# Autodesk Inventor assembly: X Axis Assembly
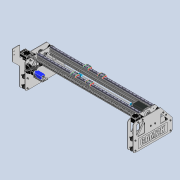
[picture p0: Inventor's stored thumbnail of the model, 180x180]
Saved by Autodesk Inventor 2022 (Build 260153000, 153)
## iProperties
Created: 2021-10-14
Part Number: X Axis Assembly
Document SubType Name: Assembly
Designer: Coy
Author: Coy
## Documents named in this file (35)
- H:\3D Files\Project 3D Models\Breakfast Maker 2000\Assemblys\X Axis Assembly.iam
- H:\3D Files\Project 3D Models\Breakfast Maker 2000\Aluminum Extrusion\2040\2040x700 silver profile.ipt
- H:\3D Files\Project 3D Models\Breakfast Maker 2000\Motors\Nema 23 Dual Shaft 87mm Stepper Motor.ipt
- H:\3D Files\Project 3D Models\Breakfast Maker 2000\Couplers\M6.35 Rigid Coupler.ipt
- H:\3D Files\Project 3D Models\Breakfast Maker 2000\Shafts and Rods\M6.35 x 356mm Aluminum Rod.ipt
- H:\3D Files\Project 3D Models\Breakfast Maker 2000\Linear Actuators\MGN12C Linear Rail.iam
- H:\3D Files\Downloaded 3D Files\GrabCad Downloads\hiwin-mgn-series-full-2.snapshot.14\PRODUCT_NAME_10.ipt
- H:\3D Files\Project 3D Models\Breakfast Maker 2000\Pullys\M6.35 24Tooth 15mm Deep 3M Timing Pulley.ipt
- H:\3D Files\Project 3D Models\Breakfast Maker 2000\Shafts and Rods\M5 55mm Threaded Rod.ipt
- H:\3D Files\Project 3D Models\Breakfast Maker 2000\Nuts and Bolts\M5 Nut Silver.ipt
- H:\3D Files\Project 3D Models\Breakfast Maker 2000\3D Printed Parts\Idler Pully Spacer.ipt
- H:\3D Files\Project 3D Models\Breakfast Maker 2000\3D Printed Parts\V Wheel Spacer.ipt
- H:\3D Files\Project 3D Models\Breakfast Maker 2000\M5 V Wheel.ipt
- H:\3D Files\Project 3D Models\Breakfast Maker 2000\Pullys\8mm ID 15mm Deep Idler Pully.ipt
- H:\3D Files\Project 3D Models\Breakfast Maker 2000\Bearings\5mm ID 8mm OD 2.5mm Deep Roller Bearing (2021_08_15 23_37_01 UTC).ipt
- H:\3D Files\Project 3D Models\Breakfast Maker 2000\3D Printed Parts\X Axis Belt and V Wheel Plate Spacer.ipt
- H:\3D Files\Project 3D Models\Breakfast Maker 2000\Bearings\0.5in Flanged Pillowblock Frame.ipt
- H:\3D Files\Project 3D Models\Breakfast Maker 2000\Bearings\0.25in ID 0.5in OD 0.1875in Deep Roller Bearing.ipt
- H:\3D Files\Project 3D Models\Breakfast Maker 2000\Machined Parts\X Axis Belt V Wheel and Motor Frame Machined.ipt
- H:\3D Files\Project 3D Models\Breakfast Maker 2000\Machined Parts\X Axis Belt V Wheel Frame Machined.ipt
- H:\3D Files\Project 3D Models\Breakfast Maker 2000\Machined Parts\X Axis Belt V Wheel LEFT Outside Frame Machined.ipt
- H:\3D Files\Project 3D Models\Breakfast Maker 2000\Machined Parts\X Axis Belt V Wheel RIGHT Outside Frame Machined.ipt
- H:\3D Files\Project 3D Models\Breakfast Maker 2000\3D Printed Parts\Y Axis Belt Stationary and Plate Spacer.ipt
- H:\3D Files\Project 3D Models\Breakfast Maker 2000\3D Printed Parts\Y Axis Belt Stationary Top.ipt
- H:\3D Files\Project 3D Models\Breakfast Maker 2000\3D Printed Parts\Y Axis Belt Adjustable and Plate Spacer.ipt
- H:\3D Files\Project 3D Models\Breakfast Maker 2000\3D Printed Parts\Y Axis Belt Adjustable Grip Plate.ipt
- H:\3D Files\Project 3D Models\Breakfast Maker 2000\Belts\HTD 3M 780mm Open End Belt.ipt
- H:\3D Files\Project 3D Models\Breakfast Maker 2000\Shafts and Rods\M5 65mm Threaded Rod.ipt
- H:\3D Files\Project 3D Models\Breakfast Maker 2000\Nuts and Bolts\M5 Silver Flat Washer.ipt
- H:\3D Files\Project 3D Models\Breakfast Maker 2000\3D Printed Parts\Y Axis Belt Adjustable Top.ipt
- H:\3D Files\Project 3D Models\Breakfast Maker 2000\Sensors\High Voltage Limit Switch\High Voltage Limit Switch.ipt
- H:\3D Files\Project 3D Models\Breakfast Maker 2000\Sensors\High Voltage Limit Switch\High Voltage Limit Switch Arm.ipt
- H:\3D Files\Project 3D Models\Breakfast Maker 2000\Sensors\High Voltage Limit Switch\High Voltage Limit Switch Arm Coupler.ipt
- H:\3D Files\Project 3D Models\Breakfast Maker 2000\3D Printed Parts\Y Axis Limit Switch Mount.ipt
- H:\3D Files\Project 3D Models\Breakfast Maker 2000\Shafts and Rods\M6.35 x 291mm Aluminum Rod.ipt
## Components (196 placed, 34 different names)
1. 2040x700 silver profile:1 — Mate:1, Flush:1, Flush:2, Mate:19, Flush:3, Mate:231, Mate:234, Mate:252, Mate:253
2. 2040x700 silver profile:2 — Flush:1, Flush:2, Flush:5, Mate:232, Mate:233, Mate:251
3. Nema 23 Dual Shaft 87mm Stepper Motor:1 — Mate:11, Mate:12, Mate:14, Mate:36, Mate:38, Mate:239, Mate:240, Mate:241
4. M6.35 Rigid Coupler:1 — Mate:11, Mate:12, Mate:13
5. M6.35 Rigid Coupler:2 — Mate:15, Mate:16, Mate:358
6. M6.35 x 356mm Aluminum Rod:1 — Mate:13, Mate:14, Mate:15, Mate:16, Mate:357
7. MGN12C Linear Rail:1 [sub-assembly] — Flush:4, Flush:5, Flush:9, Mate:25, Flush:16, Mate:27, Flush:17
8. MGN12C Linear Rail:2 [sub-assembly] — Flush:16, Mate:27, Flush:17, Flush:20, Mate:29, Flush:21
9. MGN12C Linear Rail:3 [sub-assembly] — Mate:19, Flush:3, Flush:4, Flush:6, Flush:7, Flush:8, Flush:10, Mate:24, Flush:14, Mate:26, Flush:15
10. MGN12C Linear Rail:4 [sub-assembly] — Flush:14, Mate:26, Flush:15, Flush:18, Mate:28, Flush:19
11. PRODUCT_NAME_10:1 — Flush:6, Flush:7, Mate:22, Flush:11
12. PRODUCT_NAME_10:2 — Flush:8, Flush:9, Flush:12, Mate:23, Flush:13
13. PRODUCT_NAME_10:3 — Flush:12, Mate:23, Flush:13, Mate:25
14. PRODUCT_NAME_10:4 — Flush:10, Mate:22, Flush:11, Mate:24
15. PRODUCT_NAME_10:5 — Flush:20, Mate:29, Flush:21, Flush:24, Mate:31, Flush:25
16. PRODUCT_NAME_10:6 — Flush:18, Mate:28, Flush:19, Flush:22, Mate:30, Flush:23
17. PRODUCT_NAME_10:7 — Flush:24, Mate:31, Flush:25, Flush:28, Mate:33, Flush:29
18. PRODUCT_NAME_10:8 — Flush:22, Mate:30, Flush:23, Flush:26, Mate:32, Flush:27
19. PRODUCT_NAME_10:9 — Flush:26, Mate:32, Flush:27, Mate:243
20. PRODUCT_NAME_10:10 — Flush:28, Mate:33, Flush:29, Mate:242
21. M6.35 24Tooth 15mm Deep 3M Timing Pulley:1 — Mate:36, Mate:38
22. M6.35 24Tooth 15mm Deep 3M Timing Pulley:2 — Mate:254, Mate:359
23. M5 55mm Threaded Rod:1 — Flush:34, Mate:74, Mate:84, Mate:94, Mate:107, Mate:122, Mate:132, Mate:237, Mate:295
24. M5 55mm Threaded Rod:4 — Flush:36, Mate:76, Mate:244, Mate:285, Mate:291, Mate:314
25. M5 55mm Threaded Rod:5 — Flush:38, Mate:78, Mate:86, Mate:91, Mate:101, Mate:114, Mate:118, Mate:126, Mate:134, Mate:249, Flush:151, Flush:152, Mate:299
26. M5 55mm Threaded Rod:6 — Mate:79, Flush:49, Mate:87, Mate:92, Mate:100, Mate:113, Mate:119, Mate:125, Mate:135, Mate:248, Mate:300
27. M5 55mm Threaded Rod:7 — Flush:35, Mate:75, Mate:85, Mate:95, Mate:108, Mate:121, Mate:133, Mate:238, Mate:296
28. M5 55mm Threaded Rod:8 — Flush:31, Mate:71, Mate:83, Mate:90, Mate:98, Mate:112, Mate:117, Mate:124, Mate:131, Mate:247, Mate:293
29. M5 55mm Threaded Rod:9 — Flush:31, Flush:34, Flush:35, Flush:36, Flush:37, Flush:38, Mate:70, Flush:49, Mate:82, Mate:89, Mate:99, Mate:111, Mate:116, Mate:123, Mate:130, Mate:235, Flush:147, Mate:294
30. M5 55mm Threaded Rod:10 — Flush:37, Mate:77, Mate:245, Mate:292, Mate:315
31. M5 55mm Threaded Rod:11 — Flush:48, Mate:67, Mate:161, Mate:171, Mate:180, Mate:185, Mate:191, Mate:196, Mate:201, Mate:255, Flush:148, Mate:310
32. M5 55mm Threaded Rod:12 — Flush:46, Mate:65, Mate:261, Mate:283, Mate:308
33. M5 55mm Threaded Rod:13 — Flush:44, Mate:68, Mate:159, Mate:168, Mate:176, Mate:205, Mate:208, Mate:260, Mate:305
34. M5 55mm Threaded Rod:15 — Flush:40, Mate:61, Mate:157, Mate:170, Mate:179, Mate:186, Mate:189, Mate:195, Mate:199, Mate:259, Flush:149, Mate:302
35. M5 55mm Threaded Rod:16 — Flush:40, Flush:43, Flush:44, Flush:45, Flush:46, Flush:47, Flush:48, Mate:60, Mate:156, Mate:169, Mate:178, Mate:184, Mate:190, Mate:194, Mate:200, Mate:258, Mate:301
36. M5 55mm Threaded Rod:17 — Flush:47, Mate:66, Mate:160, Mate:172, Mate:181, Mate:187, Mate:192, Mate:197, Mate:202, Mate:256, Mate:309
37. M5 55mm Threaded Rod:18 — Flush:45, Mate:64, Mate:262, Mate:282, Mate:288, Mate:307
38. M5 55mm Threaded Rod:19 — Flush:43, Mate:69, Mate:158, Mate:167, Mate:175, Mate:204, Mate:207, Mate:257, Mate:306
39. M5 Nut Silver:1 — Mate:65, Flush:65
40. M5 Nut Silver:3 — Mate:66, Flush:66
41. M5 Nut Silver:4 — Mate:67, Flush:67, Mate:263
42. M5 Nut Silver:5 — Mate:68, Flush:63
43. M5 Nut Silver:6 — Mate:69, Flush:62
44. M5 Nut Silver:7 — Mate:60, Flush:59, Flush:62, Flush:63, Flush:64, Flush:65, Flush:66, Flush:67
45. M5 Nut Silver:9 — Mate:64, Flush:64, Flush:155
46. M5 Nut Silver:10 — Mate:61, Flush:59
47. M5 Nut Silver:11 — Mate:78, Flush:57, Flush:153, Flush:154
48. M5 Nut Silver:12 — Mate:76, Flush:55
49. M5 Nut Silver:13 — Mate:79, Flush:58
50. M5 Nut Silver:14 — Mate:77, Flush:56
51. M5 Nut Silver:15 — Mate:70, Flush:50, Flush:53, Flush:54, Flush:55, Flush:56, Flush:57, Flush:58, Mate:236
52. M5 Nut Silver:16 — Mate:71, Flush:50
53. M5 Nut Silver:17 — Mate:75, Flush:54
54. M5 Nut Silver:18 — Mate:74, Flush:53
55. M5 Nut Silver:21 — Mate:98, Flush:76
56. M5 Nut Silver:22 — Mate:116, Mate:120, Flush:86, Flush:87, Flush:88, Mate:127
57. M5 Nut Silver:23 — Mate:99, Mate:102, Flush:76, Flush:77, Flush:78, Mate:115
58. M5 Nut Silver:24 — Mate:118, Flush:88
59. M5 Nut Silver:25 — Mate:87, Flush:72
60. M5 Nut Silver:26 — Mate:101, Flush:77
61. M5 Nut Silver:27 — Mate:86, Flush:71
62. M5 Nut Silver:28 — Mate:100, Flush:78
63. M5 Nut Silver:29 — Mate:85, Flush:70, Mate:97
64. M5 Nut Silver:30 — Mate:84, Flush:69, Mate:96
65. M5 Nut Silver:31 — Mate:131, Flush:92
66. M5 Nut Silver:32 — Mate:135, Flush:96
67. M5 Nut Silver:33 — Mate:130, Mate:136, Flush:92, Flush:93, Flush:94, Flush:95, Flush:96
68. M5 Nut Silver:34 — Mate:134, Flush:95
69. M5 Nut Silver:35 — Mate:119, Flush:87
70. M5 Nut Silver:36 — Mate:133, Flush:94
71. M5 Nut Silver:37 — Mate:117, Flush:86
72. M5 Nut Silver:38 — Mate:132, Flush:93
73. M5 Nut Silver:49 — Mate:83, Flush:68
74. M5 Nut Silver:50 — Mate:82, Flush:68, Flush:69, Flush:70, Flush:71, Flush:72, Mate:93, Mate:250
75. M5 Nut Silver:51 — Mate:158, Flush:108, Mate:174
76. M5 Nut Silver:52 — Mate:178, Mate:183, Flush:122
77. M5 Nut Silver:53 — Mate:159, Flush:109
78. M5 Nut Silver:54 — Mate:179, Mate:182, Flush:121, Mate:188
79. M5 Nut Silver:55 — Mate:160, Flush:110
80. M5 Nut Silver:56 — Mate:180, Flush:122
81. M5 Nut Silver:57 — Mate:161, Flush:111
82. M5 Nut Silver:58 — Mate:181, Flush:121
83. M5 Nut Silver:59 — Mate:156, Flush:107, Flush:108, Flush:109, Flush:110, Flush:111, Mate:173, Mate:267
84. M5 Nut Silver:60 — Mate:157, Flush:107
85. M5 Nut Silver:61 — Mate:189, Flush:126
86. M5 Nut Silver:62 — Mate:200, Mate:203, Flush:132, Flush:133, Flush:134
87. M5 Nut Silver:63 — Mate:190, Mate:193, Flush:126, Flush:127, Flush:128, Mate:198
88. M5 Nut Silver:64 — Mate:201, Flush:133
89. M5 Nut Silver:65 — Mate:191, Flush:127
90. M5 Nut Silver:66 — Mate:202, Flush:134
91. M5 Nut Silver:67 — Mate:192, Flush:128
92. M5 Nut Silver:68 — Mate:207, Mate:209, Flush:136
93. M5 Nut Silver:69 — Mate:199, Flush:132
94. M5 Nut Silver:70 — Mate:208, Flush:136
95. Idler Pully Spacer:1 — Mate:95, Mate:97, Mate:110
96. Idler Pully Spacer:2 — Mate:94, Mate:96, Mate:109
97. Idler Pully Spacer:3 — Mate:121, Mate:128
98. Idler Pully Spacer:4 — Mate:122, Mate:129
99. Idler Pully Spacer:5 — Mate:168, Flush:119
100. Idler Pully Spacer:6 — Mate:167, Mate:174, Flush:119, Mate:177
101. Idler Pully Spacer:7 — Mate:204, Mate:206, Flush:135, Mate:209
102. Idler Pully Spacer:8 — Mate:205, Flush:135
103. V Wheel Spacer:1 — Mate:90, Flush:73
104. V Wheel Spacer:2 — Mate:89, Mate:93, Flush:73, Flush:74, Flush:75, Mate:102
105. V Wheel Spacer:3 — Mate:91, Flush:74
106. V Wheel Spacer:4 — Mate:92, Flush:75
107. V Wheel Spacer:5 — Mate:124, Flush:89
108. V Wheel Spacer:6 — Mate:126, Flush:91
109. V Wheel Spacer:7 — Mate:123, Mate:127, Flush:89, Flush:90, Flush:91, Mate:136
110. V Wheel Spacer:8 — Mate:125, Flush:90
111. V Wheel Spacer:9 — Mate:170, Flush:116, Mate:182
112. V Wheel Spacer:10 — Mate:169, Mate:173, Flush:116, Flush:117, Flush:118, Mate:183
113. V Wheel Spacer:11 — Mate:171, Flush:117
114. V Wheel Spacer:12 — Mate:195, Flush:129
115. V Wheel Spacer:13 — Mate:172, Flush:118
116. V Wheel Spacer:14 — Mate:196, Flush:130
117. V Wheel Spacer:15 — Mate:194, Mate:198, Flush:129, Flush:130, Flush:131, Mate:203
118. V Wheel Spacer:16 — Mate:197, Flush:131
119. M5 V Wheel:1 — Mate:112, Flush:84
120. M5 V Wheel:2 — Mate:114, Flush:85
121. M5 V Wheel:3 — Mate:111, Mate:115, Flush:83, Flush:84, Flush:85, Mate:120
122. M5 V Wheel:4 — Mate:113, Flush:83
123. M5 V Wheel:5 — Mate:184, Flush:123, Mate:193
124. M5 V Wheel:6 — Mate:186, Mate:188, Flush:123, Flush:124, Flush:125
125. M5 V Wheel:7 — Mate:185, Flush:124
126. M5 V Wheel:8 — Mate:187, Flush:125
127. 8mm ID 15mm Deep Idler Pully:1 — Mate:103, Flush:79, Mate:104, Flush:80
128. 8mm ID 15mm Deep Idler Pully:2 — Mate:105, Flush:81, Mate:106, Flush:82
129. 8mm ID 15mm Deep Idler Pully:3 — Mate:165, Flush:114, Mate:166, Flush:115, Flush:120
130. 8mm ID 15mm Deep Idler Pully:4 — Mate:163, Flush:112, Mate:164, Flush:113, Flush:120
131. 5mm ID 8mm OD 2.5mm Deep Roller Bearing (2021_08_15 23_37_01 UTC):1 — Mate:104, Flush:80, Mate:110
132. 5mm ID 8mm OD 2.5mm Deep Roller Bearing (2021_08_15 23_37_01 UTC):2 — Mate:106, Flush:82, Mate:107, Mate:129
133. 5mm ID 8mm OD 2.5mm Deep Roller Bearing (2021_08_15 23_37_01 UTC):3 — Mate:103, Flush:79, Mate:108, Mate:128
134. 5mm ID 8mm OD 2.5mm Deep Roller Bearing (2021_08_15 23_37_01 UTC):4 — Mate:105, Flush:81, Mate:109
135. 5mm ID 8mm OD 2.5mm Deep Roller Bearing (2021_08_15 23_37_01 UTC):5 — Mate:165, Flush:114
136. 5mm ID 8mm OD 2.5mm Deep Roller Bearing (2021_08_15 23_37_01 UTC):6 — Mate:163, Flush:112, Mate:175, Mate:206
137. 5mm ID 8mm OD 2.5mm Deep Roller Bearing (2021_08_15 23_37_01 UTC):7 — Mate:166, Flush:115, Mate:176
138. 5mm ID 8mm OD 2.5mm Deep Roller Bearing (2021_08_15 23_37_01 UTC):8 — Mate:164, Flush:113, Mate:177
139. 0.5in Flanged Pillowblock Frame:1 — Mate:230, Flush:146, Mate:264, Mate:265, Mate:266
140. 0.25in ID 0.5in OD 0.1875in Deep Roller Bearing:1 — Mate:230, Flush:146
141. X Axis Belt V Wheel and Motor Frame Machined:1 — Mate:231, Mate:232, Mate:233, Mate:234, Mate:235, Flush:147, Mate:236, Mate:237, Mate:238, Mate:239, Mate:240, Mate:241, Mate:242, Mate:243, Mate:244, Mate:245, Mate:247, Mate:248, Mate:249, Mate:250, Mate:270, Mate:271, Mate:281
142. X Axis Belt V Wheel Frame Machined:1 — Mate:251, Mate:252, Mate:253, Mate:254, Mate:255, Mate:256, Mate:257, Mate:258, Mate:259, Mate:260, Mate:261, Mate:262, Flush:148, Mate:263, Mate:264, Mate:265, Mate:266, Mate:267, Mate:268, Mate:269, Mate:284, Mate:322, Mate:348, Mate:349, Mate:350
143. M5 55mm Threaded Rod:20 — Mate:268, Flush:149, Flush:150, Mate:275, Mate:304, Mate:321
144. M5 55mm Threaded Rod:21 — Mate:269, Flush:150, Mate:274, Mate:289, Mate:303, Mate:320
145. M5 55mm Threaded Rod:22 — Mate:270, Flush:152, Mate:273, Mate:280, Mate:286, Mate:298
146. M5 55mm Threaded Rod:23 — Mate:271, Flush:151, Mate:272, Mate:279, Mate:297
147. M5 Nut Silver:71 — Mate:272, Flush:153
148. M5 Nut Silver:72 — Mate:273, Flush:154
149. M5 Nut Silver:73 — Mate:274, Flush:156
150. M5 Nut Silver:74 — Mate:275, Flush:155, Flush:156
151. X Axis Belt and V Wheel Plate Spacer:4 — Mate:279, Mate:280, Mate:281, Mate:287
152. X Axis Belt and V Wheel Plate Spacer:5 — Mate:282, Mate:283, Mate:284, Mate:313
153. X Axis Belt V Wheel LEFT Outside Frame Machined:1 — Mate:285, Mate:286, Mate:287, Mate:312, Mate:316
154. X Axis Belt V Wheel RIGHT Outside Frame Machined:1 — Mate:288, Mate:289, Mate:311, Mate:313, Mate:354, Mate:355, Mate:356
155. M5 Nut Silver:75 — Mate:309, Flush:164, Flush:165
156. M5 Nut Silver:76 — Mate:305, Flush:160, Flush:161
157. M5 Nut Silver:77 — Mate:304, Flush:159, Flush:160
158. M5 Nut Silver:78 — Mate:302, Flush:157, Flush:158
159. M5 Nut Silver:79 — Mate:301, Mate:311, Flush:157
160. M5 Nut Silver:80 — Mate:310, Flush:165
161. M5 Nut Silver:81 — Mate:308, Flush:163, Flush:164
162. M5 Nut Silver:82 — Mate:307, Flush:162, Flush:163
163. M5 Nut Silver:83 — Mate:306, Flush:161, Flush:162
164. M5 Nut Silver:84 — Mate:303, Flush:158, Flush:159
165. M5 Nut Silver:85 — Mate:299, Flush:173, Flush:174
166. M5 Nut Silver:86 — Mate:300, Flush:174
167. M5 Nut Silver:87 — Mate:297, Flush:171, Flush:172
168. M5 Nut Silver:88 — Mate:298, Flush:172, Flush:173
169. M5 Nut Silver:89 — Mate:295, Flush:169, Flush:170
170. M5 Nut Silver:90 — Mate:296, Flush:170, Flush:171
171. M5 Nut Silver:91 — Mate:292, Flush:168, Flush:169
172. M5 Nut Silver:92 — Mate:294, Mate:312, Flush:166
173. M5 Nut Silver:93 — Mate:291, Flush:167, Flush:168
174. M5 Nut Silver:94 — Mate:293, Flush:166, Flush:167
175. Y Axis Belt Stationary and Plate Spacer:1 — Mate:314, Mate:315, Mate:316, Mate:317, Mate:318, Mate:319
176. Y Axis Belt Stationary Top:1 — Mate:317, Mate:318, Mate:319
177. Y Axis Belt Adjustable and Plate Spacer:1 — Mate:320, Mate:321, Mate:322, Mate:323, Angle:1, Mate:331, Flush:178, Mate:333
178. Y Axis Belt Adjustable Grip Plate:1 — Mate:323, Angle:1, Mate:324, Mate:325, Mate:326, Mate:327, Mate:328, Angle:2, Mate:329, Mate:330, Mate:338, Mate:340, Mate:341
179. M5 Nut Silver:95 — Mate:325, Flush:177
180. M5 Nut Silver:96 — Mate:326, Mate:328, Flush:175, Flush:176, Flush:177, Angle:2
181. M5 Nut Silver:97 — Mate:324, Flush:176
182. M5 Nut Silver:98 — Mate:327, Flush:175
183. HTD 3M 780mm Open End Belt:1 — Mate:329, Mate:330, Mate:342
184. M5 65mm Threaded Rod:1 — Mate:331, Flush:178, Mate:332, Mate:334, Mate:336, Mate:337
185. M5 Silver Flat Washer:1 — Mate:332, Mate:333, Mate:335
186. M5 Nut Silver:99 — Mate:334, Mate:335
187. M5 Nut Silver:100 — Mate:337, Mate:338, Mate:339
188. M5 Nut Silver:101 — Mate:336, Mate:339
189. Y Axis Belt Adjustable Top:1 — Mate:340, Mate:341, Mate:342
190. High Voltage Limit Switch:1 — Mate:343, Mate:344, Mate:351, Mate:352, Flush:179
191. High Voltage Limit Switch Arm:1 — Mate:345, Mate:346
192. High Voltage Limit Switch Arm Coupler:1 — Mate:343, Mate:344, Mate:345, Mate:346
193. Y Axis Limit Switch Mount:1 — Mate:348, Mate:349, Mate:350, Mate:351, Mate:352, Flush:179
194. 0.5in Flanged Pillowblock Frame:2 — Mate:353, Flush:180, Mate:354, Mate:356
195. 0.25in ID 0.5in OD 0.1875in Deep Roller Bearing:2 — Mate:353, Flush:180, Mate:355
196. M6.35 x 291mm Aluminum Rod:1 — Mate:357, Mate:358, Mate:359
## Relationships (422: Mate 269, Flush 151, Angle 2)
- Mate:1: 2040x700 silver profile:1
- Flush:1: 2040x700 silver profile:1 ↔ 2040x700 silver profile:2
- Flush:2: 2040x700 silver profile:1 ↔ 2040x700 silver profile:2
- Mate:11: Nema 23 Dual Shaft 87mm Stepper Motor:1 ↔ M6.35 Rigid Coupler:1
- Mate:12 (-12.5 mm): Nema 23 Dual Shaft 87mm Stepper Motor:1 ↔ M6.35 Rigid Coupler:1
- Mate:13: M6.35 Rigid Coupler:1 ↔ M6.35 x 356mm Aluminum Rod:1
- Mate:14: Nema 23 Dual Shaft 87mm Stepper Motor:1 ↔ M6.35 x 356mm Aluminum Rod:1
- Mate:15: M6.35 Rigid Coupler:2 ↔ M6.35 x 356mm Aluminum Rod:1
- Mate:16 (-12.5 mm): M6.35 Rigid Coupler:2 ↔ M6.35 x 356mm Aluminum Rod:1
- Mate:19: 2040x700 silver profile:1 ↔ MGN12C Linear Rail:3
- Flush:3 (4 mm): 2040x700 silver profile:1 ↔ MGN12C Linear Rail:3
- Flush:4: MGN12C Linear Rail:1 ↔ MGN12C Linear Rail:3
- Flush:5 (4 mm): 2040x700 silver profile:2 ↔ MGN12C Linear Rail:1
- Flush:6: MGN12C Linear Rail:3 ↔ PRODUCT_NAME_10:1
- Flush:7: MGN12C Linear Rail:3 ↔ PRODUCT_NAME_10:1
- Flush:8: MGN12C Linear Rail:3 ↔ PRODUCT_NAME_10:2
- Flush:9: MGN12C Linear Rail:1 ↔ PRODUCT_NAME_10:2
- Flush:10: MGN12C Linear Rail:3 ↔ PRODUCT_NAME_10:4
- Mate:22: PRODUCT_NAME_10:1 ↔ PRODUCT_NAME_10:4
- Flush:11: PRODUCT_NAME_10:1 ↔ PRODUCT_NAME_10:4
- Flush:12: PRODUCT_NAME_10:2 ↔ PRODUCT_NAME_10:3
- Mate:23: PRODUCT_NAME_10:2 ↔ PRODUCT_NAME_10:3
- Flush:13: PRODUCT_NAME_10:2 ↔ PRODUCT_NAME_10:3
- Mate:24: MGN12C Linear Rail:3 ↔ PRODUCT_NAME_10:4
- Mate:25: MGN12C Linear Rail:1 ↔ PRODUCT_NAME_10:3
- Flush:14: MGN12C Linear Rail:3 ↔ MGN12C Linear Rail:4
- Mate:26: MGN12C Linear Rail:3 ↔ MGN12C Linear Rail:4
- Flush:15: MGN12C Linear Rail:3 ↔ MGN12C Linear Rail:4
- Flush:16: MGN12C Linear Rail:1 ↔ MGN12C Linear Rail:2
- Mate:27: MGN12C Linear Rail:1 ↔ MGN12C Linear Rail:2
- Flush:17: MGN12C Linear Rail:1 ↔ MGN12C Linear Rail:2
- Flush:18: MGN12C Linear Rail:4 ↔ PRODUCT_NAME_10:6
- Mate:28: MGN12C Linear Rail:4 ↔ PRODUCT_NAME_10:6
- Flush:19: MGN12C Linear Rail:4 ↔ PRODUCT_NAME_10:6
- Flush:20: MGN12C Linear Rail:2 ↔ PRODUCT_NAME_10:5
- Mate:29: MGN12C Linear Rail:2 ↔ PRODUCT_NAME_10:5
- Flush:21: MGN12C Linear Rail:2 ↔ PRODUCT_NAME_10:5
- Flush:22: PRODUCT_NAME_10:6 ↔ PRODUCT_NAME_10:8
- Mate:30: PRODUCT_NAME_10:6 ↔ PRODUCT_NAME_10:8
- Flush:23: PRODUCT_NAME_10:6 ↔ PRODUCT_NAME_10:8
- Flush:24: PRODUCT_NAME_10:5 ↔ PRODUCT_NAME_10:7
- Mate:31: PRODUCT_NAME_10:5 ↔ PRODUCT_NAME_10:7
- Flush:25: PRODUCT_NAME_10:5 ↔ PRODUCT_NAME_10:7
- Flush:26: PRODUCT_NAME_10:8 ↔ PRODUCT_NAME_10:9
- Mate:32: PRODUCT_NAME_10:8 ↔ PRODUCT_NAME_10:9
- Flush:27: PRODUCT_NAME_10:8 ↔ PRODUCT_NAME_10:9
- Flush:28: PRODUCT_NAME_10:7 ↔ PRODUCT_NAME_10:10
- Mate:33: PRODUCT_NAME_10:7 ↔ PRODUCT_NAME_10:10
- Flush:29: PRODUCT_NAME_10:7 ↔ PRODUCT_NAME_10:10
- Mate:36: Nema 23 Dual Shaft 87mm Stepper Motor:1 ↔ M6.35 24Tooth 15mm Deep 3M Timing Pulley:1
- Mate:38 (0.15 mm): Nema 23 Dual Shaft 87mm Stepper Motor:1 ↔ M6.35 24Tooth 15mm Deep 3M Timing Pulley:1
- Flush:31: M5 55mm Threaded Rod:8 ↔ M5 55mm Threaded Rod:9
- Flush:34: M5 55mm Threaded Rod:1 ↔ M5 55mm Threaded Rod:9
- Flush:35: M5 55mm Threaded Rod:7 ↔ M5 55mm Threaded Rod:9
- Flush:36: M5 55mm Threaded Rod:4 ↔ M5 55mm Threaded Rod:9
- Flush:37: M5 55mm Threaded Rod:9 ↔ M5 55mm Threaded Rod:10
- Flush:38: M5 55mm Threaded Rod:5 ↔ M5 55mm Threaded Rod:9
- Flush:40: M5 55mm Threaded Rod:15 ↔ M5 55mm Threaded Rod:16
- Flush:43: M5 55mm Threaded Rod:16 ↔ M5 55mm Threaded Rod:19
- Flush:44: M5 55mm Threaded Rod:13 ↔ M5 55mm Threaded Rod:16
- Flush:45: M5 55mm Threaded Rod:16 ↔ M5 55mm Threaded Rod:18
- Flush:46: M5 55mm Threaded Rod:12 ↔ M5 55mm Threaded Rod:16
- Flush:47: M5 55mm Threaded Rod:16 ↔ M5 55mm Threaded Rod:17
- Flush:48: M5 55mm Threaded Rod:11 ↔ M5 55mm Threaded Rod:16
- Mate:60: M5 55mm Threaded Rod:16 ↔ M5 Nut Silver:7
- Mate:61: M5 55mm Threaded Rod:15 ↔ M5 Nut Silver:10
- Mate:64: M5 55mm Threaded Rod:18 ↔ M5 Nut Silver:9
- Mate:65: M5 55mm Threaded Rod:12 ↔ M5 Nut Silver:1
- Mate:66: M5 55mm Threaded Rod:17 ↔ M5 Nut Silver:3
- Mate:67: M5 55mm Threaded Rod:11 ↔ M5 Nut Silver:4
- Mate:68: M5 55mm Threaded Rod:13 ↔ M5 Nut Silver:5
- Mate:69: M5 55mm Threaded Rod:19 ↔ M5 Nut Silver:6
- Mate:70: M5 55mm Threaded Rod:9 ↔ M5 Nut Silver:15
- Mate:71: M5 55mm Threaded Rod:8 ↔ M5 Nut Silver:16
- Mate:74: M5 55mm Threaded Rod:1 ↔ M5 Nut Silver:18
- Mate:75: M5 55mm Threaded Rod:7 ↔ M5 Nut Silver:17
- Mate:76: M5 55mm Threaded Rod:4 ↔ M5 Nut Silver:12
- Mate:77: M5 55mm Threaded Rod:10 ↔ M5 Nut Silver:14
- Mate:78: M5 55mm Threaded Rod:5 ↔ M5 Nut Silver:11
- Mate:79: M5 55mm Threaded Rod:6 ↔ M5 Nut Silver:13
- Flush:49: M5 55mm Threaded Rod:6 ↔ M5 55mm Threaded Rod:9
- Flush:50: M5 Nut Silver:15 ↔ M5 Nut Silver:16
- Flush:53: M5 Nut Silver:15 ↔ M5 Nut Silver:18
- Flush:54: M5 Nut Silver:15 ↔ M5 Nut Silver:17
- Flush:55: M5 Nut Silver:12 ↔ M5 Nut Silver:15
- Flush:56: M5 Nut Silver:14 ↔ M5 Nut Silver:15
- Flush:57: M5 Nut Silver:11 ↔ M5 Nut Silver:15
- Flush:58: M5 Nut Silver:13 ↔ M5 Nut Silver:15
- Flush:59: M5 Nut Silver:7 ↔ M5 Nut Silver:10
- Flush:62: M5 Nut Silver:6 ↔ M5 Nut Silver:7
- Flush:63: M5 Nut Silver:5 ↔ M5 Nut Silver:7
- Flush:64: M5 Nut Silver:7 ↔ M5 Nut Silver:9
- Flush:65: M5 Nut Silver:1 ↔ M5 Nut Silver:7
- Flush:66: M5 Nut Silver:3 ↔ M5 Nut Silver:7
- Flush:67: M5 Nut Silver:4 ↔ M5 Nut Silver:7
- Mate:82: M5 55mm Threaded Rod:9 ↔ M5 Nut Silver:50
- Mate:83: M5 55mm Threaded Rod:8 ↔ M5 Nut Silver:49
- Mate:84: M5 55mm Threaded Rod:1 ↔ M5 Nut Silver:30
- Mate:85: M5 55mm Threaded Rod:7 ↔ M5 Nut Silver:29
- Mate:86: M5 55mm Threaded Rod:5 ↔ M5 Nut Silver:27
- Mate:87: M5 55mm Threaded Rod:6 ↔ M5 Nut Silver:25
- Flush:68: M5 Nut Silver:49 ↔ M5 Nut Silver:50
- Flush:69: M5 Nut Silver:30 ↔ M5 Nut Silver:50
- Flush:70: M5 Nut Silver:29 ↔ M5 Nut Silver:50
- Flush:71: M5 Nut Silver:27 ↔ M5 Nut Silver:50
- Flush:72: M5 Nut Silver:25 ↔ M5 Nut Silver:50
- Mate:89: M5 55mm Threaded Rod:9 ↔ V Wheel Spacer:2
- Mate:90: M5 55mm Threaded Rod:8 ↔ V Wheel Spacer:1
- Mate:91: M5 55mm Threaded Rod:5 ↔ V Wheel Spacer:3
- Mate:92: M5 55mm Threaded Rod:6 ↔ V Wheel Spacer:4
- Mate:93: M5 Nut Silver:50 ↔ V Wheel Spacer:2
- Flush:73: V Wheel Spacer:1 ↔ V Wheel Spacer:2
- Flush:74: V Wheel Spacer:2 ↔ V Wheel Spacer:3
- Flush:75: V Wheel Spacer:2 ↔ V Wheel Spacer:4
- Mate:94: M5 55mm Threaded Rod:1 ↔ Idler Pully Spacer:2
- Mate:95: M5 55mm Threaded Rod:7 ↔ Idler Pully Spacer:1
- Mate:96: M5 Nut Silver:30 ↔ Idler Pully Spacer:2
- Mate:97: M5 Nut Silver:29 ↔ Idler Pully Spacer:1
- Mate:98: M5 55mm Threaded Rod:8 ↔ M5 Nut Silver:21
- Mate:99: M5 55mm Threaded Rod:9 ↔ M5 Nut Silver:23
- Mate:100: M5 55mm Threaded Rod:6 ↔ M5 Nut Silver:28
- Mate:101: M5 55mm Threaded Rod:5 ↔ M5 Nut Silver:26
- Mate:102: M5 Nut Silver:23 ↔ V Wheel Spacer:2
- Flush:76: M5 Nut Silver:21 ↔ M5 Nut Silver:23
- Flush:77: M5 Nut Silver:23 ↔ M5 Nut Silver:26
- Flush:78: M5 Nut Silver:23 ↔ M5 Nut Silver:28
- Mate:103: 8mm ID 15mm Deep Idler Pully:1 ↔ 5mm ID 8mm OD 2.5mm Deep Roller Bearing (2021_08_15 23_37_01 UTC):3
- Flush:79: 8mm ID 15mm Deep Idler Pully:1 ↔ 5mm ID 8mm OD 2.5mm Deep Roller Bearing (2021_08_15 23_37_01 UTC):3
- Mate:104: 8mm ID 15mm Deep Idler Pully:1 ↔ 5mm ID 8mm OD 2.5mm Deep Roller Bearing (2021_08_15 23_37_01 UTC):1
- Flush:80: 8mm ID 15mm Deep Idler Pully:1 ↔ 5mm ID 8mm OD 2.5mm Deep Roller Bearing (2021_08_15 23_37_01 UTC):1
- Mate:105: 8mm ID 15mm Deep Idler Pully:2 ↔ 5mm ID 8mm OD 2.5mm Deep Roller Bearing (2021_08_15 23_37_01 UTC):4
- Flush:81: 8mm ID 15mm Deep Idler Pully:2 ↔ 5mm ID 8mm OD 2.5mm Deep Roller Bearing (2021_08_15 23_37_01 UTC):4
- Mate:106: 8mm ID 15mm Deep Idler Pully:2 ↔ 5mm ID 8mm OD 2.5mm Deep Roller Bearing (2021_08_15 23_37_01 UTC):2
- Flush:82: 8mm ID 15mm Deep Idler Pully:2 ↔ 5mm ID 8mm OD 2.5mm Deep Roller Bearing (2021_08_15 23_37_01 UTC):2
- Mate:107: M5 55mm Threaded Rod:1 ↔ 5mm ID 8mm OD 2.5mm Deep Roller Bearing (2021_08_15 23_37_01 UTC):2
- Mate:108: M5 55mm Threaded Rod:7 ↔ 5mm ID 8mm OD 2.5mm Deep Roller Bearing (2021_08_15 23_37_01 UTC):3
- Mate:109: Idler Pully Spacer:2 ↔ 5mm ID 8mm OD 2.5mm Deep Roller Bearing (2021_08_15 23_37_01 UTC):4
- Mate:110: Idler Pully Spacer:1 ↔ 5mm ID 8mm OD 2.5mm Deep Roller Bearing (2021_08_15 23_37_01 UTC):1
- Mate:111: M5 55mm Threaded Rod:9 ↔ M5 V Wheel:3
- Mate:112: M5 55mm Threaded Rod:8 ↔ M5 V Wheel:1
- Mate:113: M5 55mm Threaded Rod:6 ↔ M5 V Wheel:4
- Mate:114: M5 55mm Threaded Rod:5 ↔ M5 V Wheel:2
- Mate:115: M5 Nut Silver:23 ↔ M5 V Wheel:3
- Flush:83: M5 V Wheel:3 ↔ M5 V Wheel:4
- Flush:84: M5 V Wheel:1 ↔ M5 V Wheel:3
- Flush:85: M5 V Wheel:2 ↔ M5 V Wheel:3
- Mate:116: M5 55mm Threaded Rod:9 ↔ M5 Nut Silver:22
- Mate:117: M5 55mm Threaded Rod:8 ↔ M5 Nut Silver:37
- Mate:118: M5 55mm Threaded Rod:5 ↔ M5 Nut Silver:24
- Mate:119: M5 55mm Threaded Rod:6 ↔ M5 Nut Silver:35
- Mate:120: M5 Nut Silver:22 ↔ M5 V Wheel:3
- Flush:86: M5 Nut Silver:22 ↔ M5 Nut Silver:37
- Flush:87: M5 Nut Silver:22 ↔ M5 Nut Silver:35
- Flush:88: M5 Nut Silver:22 ↔ M5 Nut Silver:24
- Mate:121: M5 55mm Threaded Rod:7 ↔ Idler Pully Spacer:3
- Mate:122: M5 55mm Threaded Rod:1 ↔ Idler Pully Spacer:4
- Mate:123: M5 55mm Threaded Rod:9 ↔ V Wheel Spacer:7
- Mate:124: M5 55mm Threaded Rod:8 ↔ V Wheel Spacer:5
- Mate:125: M5 55mm Threaded Rod:6 ↔ V Wheel Spacer:8
- Mate:126: M5 55mm Threaded Rod:5 ↔ V Wheel Spacer:6
- Mate:127: M5 Nut Silver:22 ↔ V Wheel Spacer:7
- Flush:89: V Wheel Spacer:5 ↔ V Wheel Spacer:7
- Flush:90: V Wheel Spacer:7 ↔ V Wheel Spacer:8
- Flush:91: V Wheel Spacer:6 ↔ V Wheel Spacer:7
- Mate:128: Idler Pully Spacer:3 ↔ 5mm ID 8mm OD 2.5mm Deep Roller Bearing (2021_08_15 23_37_01 UTC):3
- Mate:129: Idler Pully Spacer:4 ↔ 5mm ID 8mm OD 2.5mm Deep Roller Bearing (2021_08_15 23_37_01 UTC):2
- Mate:130: M5 55mm Threaded Rod:9 ↔ M5 Nut Silver:33
- Mate:131: M5 55mm Threaded Rod:8 ↔ M5 Nut Silver:31
- Mate:132: M5 55mm Threaded Rod:1 ↔ M5 Nut Silver:38
- Mate:133: M5 55mm Threaded Rod:7 ↔ M5 Nut Silver:36
- Mate:134: M5 55mm Threaded Rod:5 ↔ M5 Nut Silver:34
- Mate:135: M5 55mm Threaded Rod:6 ↔ M5 Nut Silver:32
- Mate:136: M5 Nut Silver:33 ↔ V Wheel Spacer:7
- Flush:92: M5 Nut Silver:31 ↔ M5 Nut Silver:33
- Flush:93: M5 Nut Silver:33 ↔ M5 Nut Silver:38
- Flush:94: M5 Nut Silver:33 ↔ M5 Nut Silver:36
- Flush:95: M5 Nut Silver:33 ↔ M5 Nut Silver:34
- Flush:96: M5 Nut Silver:32 ↔ M5 Nut Silver:33
- Mate:156: M5 55mm Threaded Rod:16 ↔ M5 Nut Silver:59
- Mate:157: M5 55mm Threaded Rod:15 ↔ M5 Nut Silver:60
- Mate:158: M5 55mm Threaded Rod:19 ↔ M5 Nut Silver:51
- Mate:159: M5 55mm Threaded Rod:13 ↔ M5 Nut Silver:53
- Mate:160: M5 55mm Threaded Rod:17 ↔ M5 Nut Silver:55
- Mate:161: M5 55mm Threaded Rod:11 ↔ M5 Nut Silver:57
- Flush:107: M5 Nut Silver:59 ↔ M5 Nut Silver:60
- Flush:108: M5 Nut Silver:51 ↔ M5 Nut Silver:59
- Flush:109: M5 Nut Silver:53 ↔ M5 Nut Silver:59
- Flush:110: M5 Nut Silver:55 ↔ M5 Nut Silver:59
- Flush:111: M5 Nut Silver:57 ↔ M5 Nut Silver:59
- Mate:163: 8mm ID 15mm Deep Idler Pully:4 ↔ 5mm ID 8mm OD 2.5mm Deep Roller Bearing (2021_08_15 23_37_01 UTC):6
- Flush:112: 8mm ID 15mm Deep Idler Pully:4 ↔ 5mm ID 8mm OD 2.5mm Deep Roller Bearing (2021_08_15 23_37_01 UTC):6
- Mate:164: 8mm ID 15mm Deep Idler Pully:4 ↔ 5mm ID 8mm OD 2.5mm Deep Roller Bearing (2021_08_15 23_37_01 UTC):8
- Flush:113: 8mm ID 15mm Deep Idler Pully:4 ↔ 5mm ID 8mm OD 2.5mm Deep Roller Bearing (2021_08_15 23_37_01 UTC):8
- Mate:165: 8mm ID 15mm Deep Idler Pully:3 ↔ 5mm ID 8mm OD 2.5mm Deep Roller Bearing (2021_08_15 23_37_01 UTC):5
- Flush:114: 8mm ID 15mm Deep Idler Pully:3 ↔ 5mm ID 8mm OD 2.5mm Deep Roller Bearing (2021_08_15 23_37_01 UTC):5
- Mate:166: 8mm ID 15mm Deep Idler Pully:3 ↔ 5mm ID 8mm OD 2.5mm Deep Roller Bearing (2021_08_15 23_37_01 UTC):7
- Flush:115: 8mm ID 15mm Deep Idler Pully:3 ↔ 5mm ID 8mm OD 2.5mm Deep Roller Bearing (2021_08_15 23_37_01 UTC):7
- Mate:167: M5 55mm Threaded Rod:19 ↔ Idler Pully Spacer:6
- Mate:168: M5 55mm Threaded Rod:13 ↔ Idler Pully Spacer:5
- Mate:169: M5 55mm Threaded Rod:16 ↔ V Wheel Spacer:10
- Mate:170: M5 55mm Threaded Rod:15 ↔ V Wheel Spacer:9
- Mate:171: M5 55mm Threaded Rod:11 ↔ V Wheel Spacer:11
- Mate:172: M5 55mm Threaded Rod:17 ↔ V Wheel Spacer:13
- Mate:173: M5 Nut Silver:59 ↔ V Wheel Spacer:10
- Flush:116: V Wheel Spacer:9 ↔ V Wheel Spacer:10
- Flush:117: V Wheel Spacer:10 ↔ V Wheel Spacer:11
- Flush:118: V Wheel Spacer:10 ↔ V Wheel Spacer:13
- Mate:174: M5 Nut Silver:51 ↔ Idler Pully Spacer:6
- Flush:119: Idler Pully Spacer:5 ↔ Idler Pully Spacer:6
- Mate:175: M5 55mm Threaded Rod:19 ↔ 5mm ID 8mm OD 2.5mm Deep Roller Bearing (2021_08_15 23_37_01 UTC):6
- Mate:176: M5 55mm Threaded Rod:13 ↔ 5mm ID 8mm OD 2.5mm Deep Roller Bearing (2021_08_15 23_37_01 UTC):7
- Mate:177: Idler Pully Spacer:6 ↔ 5mm ID 8mm OD 2.5mm Deep Roller Bearing (2021_08_15 23_37_01 UTC):8
- Flush:120: 8mm ID 15mm Deep Idler Pully:3 ↔ 8mm ID 15mm Deep Idler Pully:4
- Mate:178: M5 55mm Threaded Rod:16 ↔ M5 Nut Silver:52
- Mate:179: M5 55mm Threaded Rod:15 ↔ M5 Nut Silver:54
- Mate:180: M5 55mm Threaded Rod:11 ↔ M5 Nut Silver:56
- Mate:181: M5 55mm Threaded Rod:17 ↔ M5 Nut Silver:58
- Mate:182: M5 Nut Silver:54 ↔ V Wheel Spacer:9
- Mate:183: M5 Nut Silver:52 ↔ V Wheel Spacer:10
- Flush:121: M5 Nut Silver:54 ↔ M5 Nut Silver:58
- Flush:122: M5 Nut Silver:52 ↔ M5 Nut Silver:56
- Mate:184: M5 55mm Threaded Rod:16 ↔ M5 V Wheel:5
- Mate:185: M5 55mm Threaded Rod:11 ↔ M5 V Wheel:7
- Mate:186: M5 55mm Threaded Rod:15 ↔ M5 V Wheel:6
- Mate:187: M5 55mm Threaded Rod:17 ↔ M5 V Wheel:8
- Mate:188: M5 Nut Silver:54 ↔ M5 V Wheel:6
- Flush:123: M5 V Wheel:5 ↔ M5 V Wheel:6
- Flush:124: M5 V Wheel:6 ↔ M5 V Wheel:7
- Flush:125: M5 V Wheel:6 ↔ M5 V Wheel:8
- Mate:189: M5 55mm Threaded Rod:15 ↔ M5 Nut Silver:61
- Mate:190: M5 55mm Threaded Rod:16 ↔ M5 Nut Silver:63
- Mate:191: M5 55mm Threaded Rod:11 ↔ M5 Nut Silver:65
- Mate:192: M5 55mm Threaded Rod:17 ↔ M5 Nut Silver:67
- Mate:193: M5 Nut Silver:63 ↔ M5 V Wheel:5
- Flush:126: M5 Nut Silver:61 ↔ M5 Nut Silver:63
- Flush:127: M5 Nut Silver:63 ↔ M5 Nut Silver:65
- Flush:128: M5 Nut Silver:63 ↔ M5 Nut Silver:67
- Mate:194: M5 55mm Threaded Rod:16 ↔ V Wheel Spacer:15
- Mate:195: M5 55mm Threaded Rod:15 ↔ V Wheel Spacer:12
- Mate:196: M5 55mm Threaded Rod:11 ↔ V Wheel Spacer:14
- Mate:197: M5 55mm Threaded Rod:17 ↔ V Wheel Spacer:16
- Mate:198: M5 Nut Silver:63 ↔ V Wheel Spacer:15
- Flush:129: V Wheel Spacer:12 ↔ V Wheel Spacer:15
- Flush:130: V Wheel Spacer:14 ↔ V Wheel Spacer:15
- Flush:131: V Wheel Spacer:15 ↔ V Wheel Spacer:16
- Mate:199: M5 55mm Threaded Rod:15 ↔ M5 Nut Silver:69
- Mate:200: M5 55mm Threaded Rod:16 ↔ M5 Nut Silver:62
- Mate:201: M5 55mm Threaded Rod:11 ↔ M5 Nut Silver:64
- Mate:202: M5 55mm Threaded Rod:17 ↔ M5 Nut Silver:66
- Mate:203: M5 Nut Silver:62 ↔ V Wheel Spacer:15
- Flush:132: M5 Nut Silver:62 ↔ M5 Nut Silver:69
- Flush:133: M5 Nut Silver:62 ↔ M5 Nut Silver:64
- Flush:134: M5 Nut Silver:62 ↔ M5 Nut Silver:66
- Mate:204: M5 55mm Threaded Rod:19 ↔ Idler Pully Spacer:7
- Mate:205: M5 55mm Threaded Rod:13 ↔ Idler Pully Spacer:8
- Mate:206: Idler Pully Spacer:7 ↔ 5mm ID 8mm OD 2.5mm Deep Roller Bearing (2021_08_15 23_37_01 UTC):6
- Flush:135: Idler Pully Spacer:7 ↔ Idler Pully Spacer:8
- Mate:207: M5 55mm Threaded Rod:19 ↔ M5 Nut Silver:68
- Mate:208: M5 55mm Threaded Rod:13 ↔ M5 Nut Silver:70
- Mate:209: M5 Nut Silver:68 ↔ Idler Pully Spacer:7
- Flush:136: M5 Nut Silver:68 ↔ M5 Nut Silver:70
- Mate:230: 0.5in Flanged Pillowblock Frame:1 ↔ 0.25in ID 0.5in OD 0.1875in Deep Roller Bearing:1
- Flush:146: 0.5in Flanged Pillowblock Frame:1 ↔ 0.25in ID 0.5in OD 0.1875in Deep Roller Bearing:1
- Mate:231: 2040x700 silver profile:1 ↔ X Axis Belt V Wheel and Motor Frame Machined:1
- Mate:232: 2040x700 silver profile:2 ↔ X Axis Belt V Wheel and Motor Frame Machined:1
- Mate:233: 2040x700 silver profile:2 ↔ X Axis Belt V Wheel and Motor Frame Machined:1
- Mate:234: 2040x700 silver profile:1 ↔ X Axis Belt V Wheel and Motor Frame Machined:1
- Mate:235: M5 55mm Threaded Rod:9 ↔ X Axis Belt V Wheel and Motor Frame Machined:1
- Flush:147 (-10 mm): M5 55mm Threaded Rod:9 ↔ X Axis Belt V Wheel and Motor Frame Machined:1
- Mate:236: M5 Nut Silver:15 ↔ X Axis Belt V Wheel and Motor Frame Machined:1
- Mate:237: M5 55mm Threaded Rod:1 ↔ X Axis Belt V Wheel and Motor Frame Machined:1
- Mate:238: M5 55mm Threaded Rod:7 ↔ X Axis Belt V Wheel and Motor Frame Machined:1
- Mate:239: Nema 23 Dual Shaft 87mm Stepper Motor:1 ↔ X Axis Belt V Wheel and Motor Frame Machined:1
- Mate:240: Nema 23 Dual Shaft 87mm Stepper Motor:1 ↔ X Axis Belt V Wheel and Motor Frame Machined:1
- Mate:241: Nema 23 Dual Shaft 87mm Stepper Motor:1 ↔ X Axis Belt V Wheel and Motor Frame Machined:1
- Mate:242: PRODUCT_NAME_10:10 ↔ X Axis Belt V Wheel and Motor Frame Machined:1
- Mate:243: PRODUCT_NAME_10:9 ↔ X Axis Belt V Wheel and Motor Frame Machined:1
- Mate:244: M5 55mm Threaded Rod:4 ↔ X Axis Belt V Wheel and Motor Frame Machined:1
- Mate:245: M5 55mm Threaded Rod:10 ↔ X Axis Belt V Wheel and Motor Frame Machined:1
- Mate:247: M5 55mm Threaded Rod:8 ↔ X Axis Belt V Wheel and Motor Frame Machined:1
- Mate:248: M5 55mm Threaded Rod:6 ↔ X Axis Belt V Wheel and Motor Frame Machined:1
- Mate:249: M5 55mm Threaded Rod:5 ↔ X Axis Belt V Wheel and Motor Frame Machined:1
- Mate:250: M5 Nut Silver:50 ↔ X Axis Belt V Wheel and Motor Frame Machined:1
- Mate:251: 2040x700 silver profile:2 ↔ X Axis Belt V Wheel Frame Machined:1
- Mate:252: 2040x700 silver profile:1 ↔ X Axis Belt V Wheel Frame Machined:1
- Mate:253: 2040x700 silver profile:1 ↔ X Axis Belt V Wheel Frame Machined:1
- Mate:254 (4.575 mm): M6.35 24Tooth 15mm Deep 3M Timing Pulley:2 ↔ X Axis Belt V Wheel Frame Machined:1
- Mate:255: M5 55mm Threaded Rod:11 ↔ X Axis Belt V Wheel Frame Machined:1
- Mate:256: M5 55mm Threaded Rod:17 ↔ X Axis Belt V Wheel Frame Machined:1
- Mate:257: M5 55mm Threaded Rod:19 ↔ X Axis Belt V Wheel Frame Machined:1
- Mate:258: M5 55mm Threaded Rod:16 ↔ X Axis Belt V Wheel Frame Machined:1
- Mate:259: M5 55mm Threaded Rod:15 ↔ X Axis Belt V Wheel Frame Machined:1
- Mate:260: M5 55mm Threaded Rod:13 ↔ X Axis Belt V Wheel Frame Machined:1
- Mate:261: M5 55mm Threaded Rod:12 ↔ X Axis Belt V Wheel Frame Machined:1
- Mate:262: M5 55mm Threaded Rod:18 ↔ X Axis Belt V Wheel Frame Machined:1
- Flush:148 (-10 mm): M5 55mm Threaded Rod:11 ↔ X Axis Belt V Wheel Frame Machined:1
- Mate:263: M5 Nut Silver:4 ↔ X Axis Belt V Wheel Frame Machined:1
- Mate:264: 0.5in Flanged Pillowblock Frame:1 ↔ X Axis Belt V Wheel Frame Machined:1
- Mate:265: 0.5in Flanged Pillowblock Frame:1 ↔ X Axis Belt V Wheel Frame Machined:1
- Mate:266: 0.5in Flanged Pillowblock Frame:1 ↔ X Axis Belt V Wheel Frame Machined:1
- Mate:267: M5 Nut Silver:59 ↔ X Axis Belt V Wheel Frame Machined:1
- Mate:268: X Axis Belt V Wheel Frame Machined:1 ↔ M5 55mm Threaded Rod:20
- Mate:269: X Axis Belt V Wheel Frame Machined:1 ↔ M5 55mm Threaded Rod:21
- Mate:270: X Axis Belt V Wheel and Motor Frame Machined:1 ↔ M5 55mm Threaded Rod:22
- Mate:271: X Axis Belt V Wheel and Motor Frame Machined:1 ↔ M5 55mm Threaded Rod:23
- Flush:149: M5 55mm Threaded Rod:15 ↔ M5 55mm Threaded Rod:20
- Flush:150: M5 55mm Threaded Rod:20 ↔ M5 55mm Threaded Rod:21
- Flush:151: M5 55mm Threaded Rod:5 ↔ M5 55mm Threaded Rod:23
- Flush:152: M5 55mm Threaded Rod:5 ↔ M5 55mm Threaded Rod:22
- Mate:272: M5 55mm Threaded Rod:23 ↔ M5 Nut Silver:71
- Mate:273: M5 55mm Threaded Rod:22 ↔ M5 Nut Silver:72
- Flush:153: M5 Nut Silver:11 ↔ M5 Nut Silver:71
- Flush:154: M5 Nut Silver:11 ↔ M5 Nut Silver:72
- Mate:274: M5 55mm Threaded Rod:21 ↔ M5 Nut Silver:73
- Mate:275: M5 55mm Threaded Rod:20 ↔ M5 Nut Silver:74
- Flush:155: M5 Nut Silver:9 ↔ M5 Nut Silver:74
- Flush:156: M5 Nut Silver:73 ↔ M5 Nut Silver:74
- Mate:279: M5 55mm Threaded Rod:23 ↔ X Axis Belt and V Wheel Plate Spacer:4
- Mate:280: M5 55mm Threaded Rod:22 ↔ X Axis Belt and V Wheel Plate Spacer:4
- Mate:281: X Axis Belt V Wheel and Motor Frame Machined:1 ↔ X Axis Belt and V Wheel Plate Spacer:4
- Mate:282: M5 55mm Threaded Rod:18 ↔ X Axis Belt and V Wheel Plate Spacer:5
- Mate:283: M5 55mm Threaded Rod:12 ↔ X Axis Belt and V Wheel Plate Spacer:5
- Mate:284: X Axis Belt V Wheel Frame Machined:1 ↔ X Axis Belt and V Wheel Plate Spacer:5
- Mate:285: M5 55mm Threaded Rod:4 ↔ X Axis Belt V Wheel LEFT Outside Frame Machined:1
- Mate:286: M5 55mm Threaded Rod:22 ↔ X Axis Belt V Wheel LEFT Outside Frame Machined:1
- Mate:287: X Axis Belt and V Wheel Plate Spacer:4 ↔ X Axis Belt V Wheel LEFT Outside Frame Machined:1
- Mate:288: M5 55mm Threaded Rod:18 ↔ X Axis Belt V Wheel RIGHT Outside Frame Machined:1
- Mate:289: M5 55mm Threaded Rod:21 ↔ X Axis Belt V Wheel RIGHT Outside Frame Machined:1
- Mate:291: M5 55mm Threaded Rod:4 ↔ M5 Nut Silver:93
- Mate:292: M5 55mm Threaded Rod:10 ↔ M5 Nut Silver:91
- Mate:293: M5 55mm Threaded Rod:8 ↔ M5 Nut Silver:94
- Mate:294: M5 55mm Threaded Rod:9 ↔ M5 Nut Silver:92
- Mate:295: M5 55mm Threaded Rod:1 ↔ M5 Nut Silver:89
- Mate:296: M5 55mm Threaded Rod:7 ↔ M5 Nut Silver:90
- Mate:297: M5 55mm Threaded Rod:23 ↔ M5 Nut Silver:87
- Mate:298: M5 55mm Threaded Rod:22 ↔ M5 Nut Silver:88
- Mate:299: M5 55mm Threaded Rod:5 ↔ M5 Nut Silver:85
- Mate:300: M5 55mm Threaded Rod:6 ↔ M5 Nut Silver:86
- Mate:301: M5 55mm Threaded Rod:16 ↔ M5 Nut Silver:79
- Mate:302: M5 55mm Threaded Rod:15 ↔ M5 Nut Silver:78
- Mate:303: M5 55mm Threaded Rod:21 ↔ M5 Nut Silver:84
- Mate:304: M5 55mm Threaded Rod:20 ↔ M5 Nut Silver:77
- Mate:305: M5 55mm Threaded Rod:13 ↔ M5 Nut Silver:76
- Mate:306: M5 55mm Threaded Rod:19 ↔ M5 Nut Silver:83
- Mate:307: M5 55mm Threaded Rod:18 ↔ M5 Nut Silver:82
- Mate:308: M5 55mm Threaded Rod:12 ↔ M5 Nut Silver:81
- Mate:309: M5 55mm Threaded Rod:17 ↔ M5 Nut Silver:75
- Mate:310: M5 55mm Threaded Rod:11 ↔ M5 Nut Silver:80
- Mate:311: X Axis Belt V Wheel RIGHT Outside Frame Machined:1 ↔ M5 Nut Silver:79
- Flush:157: M5 Nut Silver:78 ↔ M5 Nut Silver:79
- Flush:158: M5 Nut Silver:78 ↔ M5 Nut Silver:84
- Flush:159: M5 Nut Silver:77 ↔ M5 Nut Silver:84
- Flush:160: M5 Nut Silver:76 ↔ M5 Nut Silver:77
- Flush:161: M5 Nut Silver:76 ↔ M5 Nut Silver:83
- Flush:162: M5 Nut Silver:82 ↔ M5 Nut Silver:83
- Flush:163: M5 Nut Silver:81 ↔ M5 Nut Silver:82
- Flush:164: M5 Nut Silver:75 ↔ M5 Nut Silver:81
- Flush:165: M5 Nut Silver:75 ↔ M5 Nut Silver:80
- Mate:312: X Axis Belt V Wheel LEFT Outside Frame Machined:1 ↔ M5 Nut Silver:92
- Flush:166: M5 Nut Silver:92 ↔ M5 Nut Silver:94
- Flush:167: M5 Nut Silver:93 ↔ M5 Nut Silver:94
- Flush:168: M5 Nut Silver:91 ↔ M5 Nut Silver:93
- Flush:169: M5 Nut Silver:89 ↔ M5 Nut Silver:91
- Flush:170: M5 Nut Silver:89 ↔ M5 Nut Silver:90
- Flush:171: M5 Nut Silver:87 ↔ M5 Nut Silver:90
- Flush:172: M5 Nut Silver:87 ↔ M5 Nut Silver:88
- Flush:173: M5 Nut Silver:85 ↔ M5 Nut Silver:88
- Flush:174: M5 Nut Silver:85 ↔ M5 Nut Silver:86
- Mate:313: X Axis Belt and V Wheel Plate Spacer:5 ↔ X Axis Belt V Wheel RIGHT Outside Frame Machined:1
- Mate:314: M5 55mm Threaded Rod:4 ↔ Y Axis Belt Stationary and Plate Spacer:1
- Mate:315: M5 55mm Threaded Rod:10 ↔ Y Axis Belt Stationary and Plate Spacer:1
- Mate:316: X Axis Belt V Wheel LEFT Outside Frame Machined:1 ↔ Y Axis Belt Stationary and Plate Spacer:1
- Mate:317: Y Axis Belt Stationary and Plate Spacer:1 ↔ Y Axis Belt Stationary Top:1
- Mate:318: Y Axis Belt Stationary and Plate Spacer:1 ↔ Y Axis Belt Stationary Top:1
- Mate:319 (2.4 mm): Y Axis Belt Stationary and Plate Spacer:1 ↔ Y Axis Belt Stationary Top:1
- Mate:320: M5 55mm Threaded Rod:21 ↔ Y Axis Belt Adjustable and Plate Spacer:1
- Mate:321: M5 55mm Threaded Rod:20 ↔ Y Axis Belt Adjustable and Plate Spacer:1
- Mate:322: X Axis Belt V Wheel Frame Machined:1 ↔ Y Axis Belt Adjustable and Plate Spacer:1
- Mate:323: Y Axis Belt Adjustable and Plate Spacer:1 ↔ Y Axis Belt Adjustable Grip Plate:1
- Angle:1 (0 deg): Y Axis Belt Adjustable and Plate Spacer:1 ↔ Y Axis Belt Adjustable Grip Plate:1
- Mate:324: Y Axis Belt Adjustable Grip Plate:1 ↔ M5 Nut Silver:97
- Mate:325: Y Axis Belt Adjustable Grip Plate:1 ↔ M5 Nut Silver:95
- Mate:326: Y Axis Belt Adjustable Grip Plate:1 ↔ M5 Nut Silver:96
- Mate:327: Y Axis Belt Adjustable Grip Plate:1 ↔ M5 Nut Silver:98
- Mate:328: Y Axis Belt Adjustable Grip Plate:1 ↔ M5 Nut Silver:96
- Flush:175: M5 Nut Silver:96 ↔ M5 Nut Silver:98
- Flush:176: M5 Nut Silver:96 ↔ M5 Nut Silver:97
- Flush:177: M5 Nut Silver:95 ↔ M5 Nut Silver:96
- Angle:2 (0 deg): Y Axis Belt Adjustable Grip Plate:1 ↔ M5 Nut Silver:96
- Mate:329 (0.5 mm): Y Axis Belt Adjustable Grip Plate:1 ↔ HTD 3M 780mm Open End Belt:1
- Mate:330: Y Axis Belt Adjustable Grip Plate:1 ↔ HTD 3M 780mm Open End Belt:1
- Mate:331: Y Axis Belt Adjustable and Plate Spacer:1 ↔ M5 65mm Threaded Rod:1
- Flush:178 (-3 mm): Y Axis Belt Adjustable and Plate Spacer:1 ↔ M5 65mm Threaded Rod:1
- Mate:332: M5 65mm Threaded Rod:1 ↔ M5 Silver Flat Washer:1
- Mate:333: Y Axis Belt Adjustable and Plate Spacer:1 ↔ M5 Silver Flat Washer:1
- Mate:334: M5 65mm Threaded Rod:1 ↔ M5 Nut Silver:99
- Mate:335: M5 Silver Flat Washer:1 ↔ M5 Nut Silver:99
- Mate:336: M5 65mm Threaded Rod:1 ↔ M5 Nut Silver:101
- Mate:337: M5 65mm Threaded Rod:1 ↔ M5 Nut Silver:100
- Mate:338: Y Axis Belt Adjustable Grip Plate:1 ↔ M5 Nut Silver:100
- Mate:339: M5 Nut Silver:100 ↔ M5 Nut Silver:101
- Mate:340: Y Axis Belt Adjustable Grip Plate:1 ↔ Y Axis Belt Adjustable Top:1
- Mate:341: Y Axis Belt Adjustable Grip Plate:1 ↔ Y Axis Belt Adjustable Top:1
- Mate:342: HTD 3M 780mm Open End Belt:1 ↔ Y Axis Belt Adjustable Top:1
- Mate:343: High Voltage Limit Switch:1 ↔ High Voltage Limit Switch Arm Coupler:1
- Mate:344 (1.5 mm): High Voltage Limit Switch:1 ↔ High Voltage Limit Switch Arm Coupler:1
- Mate:345: High Voltage Limit Switch Arm:1 ↔ High Voltage Limit Switch Arm Coupler:1
- Mate:346: High Voltage Limit Switch Arm:1 ↔ High Voltage Limit Switch Arm Coupler:1
- Mate:348: X Axis Belt V Wheel Frame Machined:1 ↔ Y Axis Limit Switch Mount:1
- Mate:349: X Axis Belt V Wheel Frame Machined:1 ↔ Y Axis Limit Switch Mount:1
- Mate:350: X Axis Belt V Wheel Frame Machined:1 ↔ Y Axis Limit Switch Mount:1
- Mate:351: High Voltage Limit Switch:1 ↔ Y Axis Limit Switch Mount:1
- Mate:352 (0.2 mm): High Voltage Limit Switch:1 ↔ Y Axis Limit Switch Mount:1
- Flush:179: High Voltage Limit Switch:1 ↔ Y Axis Limit Switch Mount:1
- Mate:353: 0.5in Flanged Pillowblock Frame:2 ↔ 0.25in ID 0.5in OD 0.1875in Deep Roller Bearing:2
- Flush:180: 0.5in Flanged Pillowblock Frame:2 ↔ 0.25in ID 0.5in OD 0.1875in Deep Roller Bearing:2
- Mate:354: X Axis Belt V Wheel RIGHT Outside Frame Machined:1 ↔ 0.5in Flanged Pillowblock Frame:2
- Mate:355: X Axis Belt V Wheel RIGHT Outside Frame Machined:1 ↔ 0.25in ID 0.5in OD 0.1875in Deep Roller Bearing:2
- Mate:356: X Axis Belt V Wheel RIGHT Outside Frame Machined:1 ↔ 0.5in Flanged Pillowblock Frame:2
- Mate:357: M6.35 x 356mm Aluminum Rod:1 ↔ M6.35 x 291mm Aluminum Rod:1
- Mate:358: M6.35 Rigid Coupler:2 ↔ M6.35 x 291mm Aluminum Rod:1
- Mate:359: M6.35 24Tooth 15mm Deep 3M Timing Pulley:2 ↔ M6.35 x 291mm Aluminum Rod:1
